# Autodesk Inventor assembly: SpindleMotor
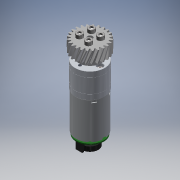
[picture p0: Inventor's stored thumbnail of the model, 180x180]
Saved by Autodesk Inventor 2018.3 (Build 223284000, 284)
## iProperties
Created: 2018-08-14
Part Number: SpindleMotor
Material: Generisch
Document SubType Name: Assembly
Designer: JochenAlt
Author: JochenAlt
## Documents named in this file (5)
- D:\Projects\Ondine\CAD\SpindleMotor.iam
- D:\Projects\Ondine\CAD\Mounting Hub.ipt
- D:\Projects\Ondine\CAD\Pololu Motor 25D\25D Gearmotor Unit.iam
- D:\Projects\Ondine\CAD\Spindle\Konstruktions-Assistent\Stirnzahnrad21.ipt
- C:\Users\JochenAlt\Documents\Inventor\Content Center Files\R2018\de-DE\DIN 912\DIN 912 - M3 x 0,5 x 10 x 8,75.ipt
## Components (7 placed, 4 different names)
1. Mounting Hub:1 — Passend:1, Passend:2, Passend:4
2. 25D Gearmotor Unit:1 [sub-assembly] — Passend:1, Passend:2, Passend:3
3. Stirnzahnrad2:1 — Passend:3, Passend:4, Einfügen:1, Einfügen:2, Einfügen:3, Einfügen:4
4. DIN 912 - ersetzt durch DIN EN ISO 4762 M3 x 10:1 — Einfügen:1
5. DIN 912 - ersetzt durch DIN EN ISO 4762 M3 x 10:2 — Einfügen:2
6. DIN 912 - ersetzt durch DIN EN ISO 4762 M3 x 10:3 — Einfügen:3
7. DIN 912 - ersetzt durch DIN EN ISO 4762 M3 x 10:4 — Einfügen:4
## Relationships (8: Mate 4, Insert 4)
- Passend:1 [Mate]: Mounting Hub:1 ↔ 25D Gearmotor Unit:1
- Passend:2 [Mate] (0.5 mm): Mounting Hub:1 ↔ 25D Gearmotor Unit:1
- Passend:3 [Mate]: 25D Gearmotor Unit:1 ↔ Stirnzahnrad2:1
- Passend:4 [Mate]: Mounting Hub:1 ↔ Stirnzahnrad2:1
- Einfügen:1 [Insert]: Stirnzahnrad2:1 ↔ DIN 912 - ersetzt durch DIN EN ISO 4762 M3 x 10:1
- Einfügen:2 [Insert]: Stirnzahnrad2:1 ↔ DIN 912 - ersetzt durch DIN EN ISO 4762 M3 x 10:2
- Einfügen:3 [Insert]: Stirnzahnrad2:1 ↔ DIN 912 - ersetzt durch DIN EN ISO 4762 M3 x 10:3
- Einfügen:4 [Insert]: Stirnzahnrad2:1 ↔ DIN 912 - ersetzt durch DIN EN ISO 4762 M3 x 10:4
